# Autodesk Inventor assembly: invacare assy
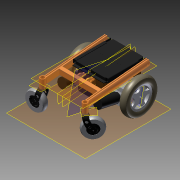
[picture p0: Inventor's stored thumbnail of the model, 180x180]
Saved by Autodesk Inventor 2012 (Build 160160000, 160)
## iProperties
Created: 2012-03-08
Part Number: invacare assy
Document SubType Name: Assembly
Designer: esv
Mass: 83979.9 g
Surface Area: 24308.3 cm^2
Volume: 48170.3 cm^3
Density: 1.7434 g/cm^3
Author: esv
## Documents named in this file (6)
- C:\Users\esv\masters\CAD\Invacare\invacare assy.iam
- C:\Users\esv\masters\CAD\Invacare\frame assy.iam
- C:\Users\esv\masters\CAD\Invacare\battery.ipt
- C:\Users\esv\masters\CAD\Invacare\motor.ipt
- C:\Users\esv\masters\CAD\Invacare\motor_MIR.ipt
- C:\Users\esv\masters\CAD\Invacare\wheel.ipt
## Components (7 placed, 5 different names)
1. frame assy:1 [sub-assembly] — Flush:1, Angle:1, Mate:2, Mate:3, Mate:4, Flush:6, Mate:10, Mate:11
2. battery:1 — Mate:1, Flush:2, Flush:3, Mate:2
3. battery:2 — Mate:1, Flush:2, Flush:3, Mate:3, Mate:4
4. motor:1 — Mate:7, Mate:8, Flush:4, Flush:5, Mate:9
5. motor_MIR:1 — Mate:5, Mate:6, Flush:4, Flush:5, Mate:9, Flush:6, Flush:7, Mate:11
6. wheel:1 — Mate:5, Mate:6
7. wheel:2 — Mate:7, Mate:8
## Relationships (19: Mate 11, Flush 7, Angle 1)
- Flush:1: frame assy:1
- Angle:1 (0 deg): frame assy:1
- Mate:1: battery:1 ↔ battery:2
- Flush:2: battery:1 ↔ battery:2
- Flush:3: battery:1 ↔ battery:2
- Mate:2: frame assy:1 ↔ battery:1
- Mate:3: frame assy:1 ↔ battery:2
- Mate:4: frame assy:1 ↔ battery:2
- Mate:5: motor_MIR:1 ↔ wheel:1
- Mate:6: motor_MIR:1 ↔ wheel:1
- Mate:7: motor:1 ↔ wheel:2
- Mate:8: motor:1 ↔ wheel:2
- Flush:4: motor:1 ↔ motor_MIR:1
- Flush:5: motor:1 ↔ motor_MIR:1
- Mate:9 (285.75 mm): motor:1 ↔ motor_MIR:1
- Flush:6 (233.3625 mm): frame assy:1 ↔ motor_MIR:1
- Flush:7 (142.875 mm): motor_MIR:1
- Mate:10: frame assy:1
- Mate:11 (-101.6 mm): frame assy:1 ↔ motor_MIR:1
